# Autodesk Inventor assembly: A2017_T3_02
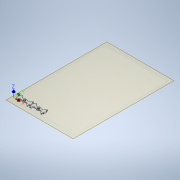
[picture p0: Inventor's stored thumbnail of the model, 180x180]
Saved by Autodesk Inventor 2020 (Build 240168000, 168)
## iProperties
Created: 2021-08-27
Part Number: A2017_T3_02
Document SubType Name: Assembly
Designer: Masato
Author: Masato
## Documents named in this file (3)
- C:\Users\naoki\Documents\Inventor\CitBrains\git_clone\OpenPlatform4_1\コックピット\OpenPlatform_ver3_0\cam\A2017_T3_02.iam
- C:\Users\naoki\Documents\Inventor\CitBrains\git_clone\OpenPlatform4_1\コックピット\OpenPlatform_ver3_0\cam\Disposable_Board.ipt
- C:\Users\naoki\Documents\Inventor\CitBrains\git_clone\OpenPlatform4_1\コックピット\OpenPlatform_ver3_0\LowerBody\Ankle\Ankle_front_frame.ipt
## Components (3 placed, 2 different names)
1. Disposable_Board:1 — メイト:2, メイト:1, フラッシュ:1, フラッシュ:2, メイト:4, フラッシュ:3, フラッシュ:4
2. Ankle_front_frame:1 — メイト:4, フラッシュ:3, フラッシュ:4
3. Ankle_front_frame:2
## Component patterns: (2 elements, first: Ankle_front_frame:1)
## Relationships (7: Flush 4, Mate 3)
- メイト:2 [Mate]: Disposable_Board:1
- メイト:1 [Mate]: Disposable_Board:1
- フラッシュ:1 [Flush]: Disposable_Board:1
- フラッシュ:2 [Flush]: Disposable_Board:1
- メイト:4 [Mate]: Disposable_Board:1 ↔ Ankle_front_frame:1
- フラッシュ:3 [Flush] (2 mm): Disposable_Board:1 ↔ Ankle_front_frame:1
- フラッシュ:4 [Flush] (2 mm): Disposable_Board:1 ↔ Ankle_front_frame:1
